# Autodesk Inventor assembly: MOGO Funnel
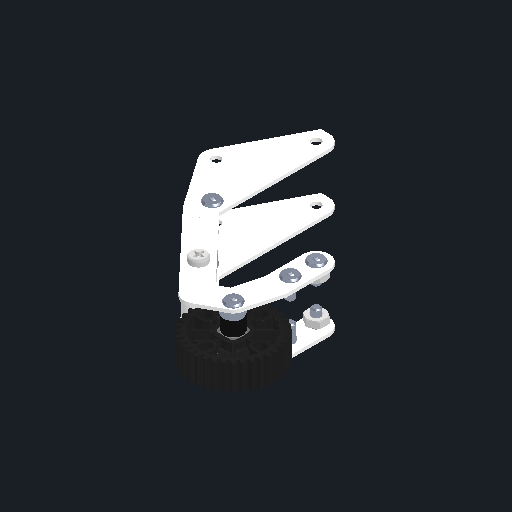
[picture p0: Inventor's stored thumbnail of the model, 512x512]
Saved by Autodesk Inventor 2025 (Build 290162000, 162)
## iProperties
Created: 2024-12-17
Part Number: MOGO Funnel
Document SubType Name: Assembly
Designer: Averey Ku
Author: Averey Ku
## Documents named in this file (18)
- D:\VEX\High Stakes\CAD\V4\Chassis\Drivebay Right\MOGO Funnel.iam
- D:\VEX\High Stakes\CAD\V4\Chassis\Drivebay Right\Ring Funnel1.ipt
- D:\VEX\High Stakes\CAD\ROBOPROS-CAD-Inventor\Motion\Spacers\Spacer Nylon .375 OD.ipt
- D:\VEX\High Stakes\CAD\ROBOPROS-CAD-Inventor\Motion\Spacers\Spacer Nylon .500 OD\NSpacer White .500 OD x .500.ipt
- D:\VEX\High Stakes\CAD\ROBOPROS-CAD-Inventor\Motion\Spacers\Spacer Nylon .500 OD.ipt
- D:\VEX\High Stakes\CAD\V4\Chassis\Drivebay Right\HS 36T Gear, No Insert1.iam
- D:\VEX\High Stakes\CAD\V4\Chassis\Drivebay Right\NScrew Pan Head Threaded 1.2501.ipt
- D:\VEX\High Stakes\CAD\ROBOPROS-CAD-Inventor\Structure\Hardware\Screw Steel - Star\SScrew Star Smooth 1.250.ipt
- D:\VEX\High Stakes\CAD\ROBOPROS-CAD-Inventor\Structure\Hardware\Screw Steel - Star.ipt
- D:\VEX\High Stakes\CAD\V4\Chassis\Drivebay Right\Nut Nylon Thread-Forming1.ipt
- D:\VEX\High Stakes\CAD\ROBOPROS-CAD-Inventor\Structure\Hardware\Screw Shoulder Robosource\SScrew Shoulder Smooth .375 x .12.ipt
- D:\VEX\High Stakes\CAD\ROBOPROS-CAD-Inventor\Structure\Hardware\Screw Shoulder Robosource.ipt
- D:\VEX\High Stakes\CAD\ROBOPROS-CAD-Inventor\Motion\Spacers\Washer Steel\SWasher .375 OD x .062500.ipt
- D:\VEX\High Stakes\CAD\ROBOPROS-CAD-Inventor\Motion\Spacers\Washer Steel.ipt
- D:\VEX\High Stakes\CAD\ROBOPROS-CAD-Inventor\Motion\Spacers\Washer Steel\SWasher .375 OD x .031250.ipt
- D:\VEX\High Stakes\CAD\V4\Chassis\Drivebay Right\Nut Keps1.ipt
- D:\VEX\High Stakes\CAD\ROBOPROS-CAD-Inventor\Motion\Spacers\Spacer Nylon .375 OD\NSpacer .375 OD x .250.ipt
- D:\VEX\High Stakes\CAD\V4\Chassis\Drivebay Right\MOGO Funnel.ipt
## Components (25 placed, 12 different names)
1. Ring Funnel1:1 — Insert:1, Mate:1, Insert:5, Insert:9, Insert:11, Insert:19, Insert:17, Insert:18, Insert:23, Insert:27, Mate:2, Insert:30
2. Ring Funnel1:2 — Insert:1, Mate:1, Insert:6, Insert:13, Insert:15, Insert:16, Insert:21, Insert:20, Insert:22, Insert:24, Insert:26, Mate:3, Insert:31
3. NSpacer White .500 OD x .500:1 — Insert:4
4. NSpacer White .500 OD x .500:2 — Insert:4, Insert:5
5. HS 36T Gear, No Insert1:1 [sub-assembly] — Insert:6
6. NScrew Pan Head Threaded 1.2501:1 — Insert:9
7. SScrew Star Smooth 1.250:1 — Insert:11
8. Nut Nylon Thread-Forming1:1 — Insert:13
9. Nut Nylon Thread-Forming1:2 — Insert:15
10. Nut Nylon Thread-Forming1:3 — Insert:16
11. SScrew Shoulder Smooth .375 x .12:1 — Insert:19
12. SScrew Shoulder Smooth .375 x .12:2 — Insert:17
13. SScrew Shoulder Smooth .375 x .12:3 — Insert:18
14. SScrew Shoulder Smooth .375 x .12:4 — Insert:21
15. SScrew Shoulder Smooth .375 x .12:5 — Insert:20
16. SScrew Shoulder Smooth .375 x .12:6 — Insert:22
17. Nut Nylon Thread-Forming1:4 — Insert:23
18. Nut Nylon Thread-Forming1:5 — Insert:24
19. SWasher .375 OD x .062500:1 — Insert:26, Insert:25
20. SWasher .375 OD x .031250:2 — Insert:25
21. Nut Keps1:1 — Insert:27, Insert:29
22. SWasher .375 OD x .062500:3 — Insert:28
23. NSpacer .375 OD x .250:3 — Insert:28, Insert:29
24. MOGO Funnel:1 — Mate:2, Insert:30
25. MOGO Funnel:2 — Mate:3, Insert:31
## Relationships (27: Insert 24, Mate 3)
- Insert:1 (25.4 mm): Ring Funnel1:1 ↔ Ring Funnel1:2
- Mate:1: Ring Funnel1:1 ↔ Ring Funnel1:2
- Insert:4: NSpacer White .500 OD x .500:1 ↔ NSpacer White .500 OD x .500:2
- Insert:5: Ring Funnel1:1 ↔ NSpacer White .500 OD x .500:2
- Insert:6 (2.3813 mm): Ring Funnel1:2 ↔ HS 36T Gear, No Insert1:1
- Insert:9: Ring Funnel1:1 ↔ NScrew Pan Head Threaded 1.2501:1
- Insert:11: Ring Funnel1:1 ↔ SScrew Star Smooth 1.250:1
- Insert:13: Ring Funnel1:2 ↔ Nut Nylon Thread-Forming1:1
- Insert:15: Ring Funnel1:2 ↔ Nut Nylon Thread-Forming1:2
- Insert:16: Ring Funnel1:2 ↔ Nut Nylon Thread-Forming1:3
- Insert:19: Ring Funnel1:1 ↔ SScrew Shoulder Smooth .375 x .12:1
- Insert:17: Ring Funnel1:1 ↔ SScrew Shoulder Smooth .375 x .12:2
- Insert:18: Ring Funnel1:1 ↔ SScrew Shoulder Smooth .375 x .12:3
- Insert:21: Ring Funnel1:2 ↔ SScrew Shoulder Smooth .375 x .12:4
- Insert:20: Ring Funnel1:2 ↔ SScrew Shoulder Smooth .375 x .12:5
- Insert:22: Ring Funnel1:2 ↔ SScrew Shoulder Smooth .375 x .12:6
- Insert:23 (1.5875 mm): Ring Funnel1:1 ↔ Nut Nylon Thread-Forming1:4
- Insert:24 (1.5875 mm): Ring Funnel1:2 ↔ Nut Nylon Thread-Forming1:5
- Insert:26: Ring Funnel1:2 ↔ SWasher .375 OD x .062500:1
- Insert:25: SWasher .375 OD x .062500:1 ↔ SWasher .375 OD x .031250:2
- Insert:27: Ring Funnel1:1 ↔ Nut Keps1:1
- Insert:28: SWasher .375 OD x .062500:3 ↔ NSpacer .375 OD x .250:3
- Insert:29: Nut Keps1:1 ↔ NSpacer .375 OD x .250:3
- Mate:2: Ring Funnel1:1 ↔ MOGO Funnel:1
- Insert:30: Ring Funnel1:1 ↔ MOGO Funnel:1
- Mate:3: Ring Funnel1:2 ↔ MOGO Funnel:2
- Insert:31: Ring Funnel1:2 ↔ MOGO Funnel:2
